# Autodesk Inventor assembly: kls15-225-m12
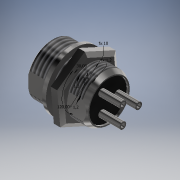
[picture p0: Inventor's stored thumbnail of the model, 180x180]
Saved by Autodesk Inventor 2019 (Build 230136000, 136)
## iProperties
Created: 2019-07-16
Part Number: kls15-225-m12
Material: Типовые
Document SubType Name: Assembly
Designer: Boss
Mass: 8.12231 g
Surface Area: 21.6045 cm^2
Volume: 1.41247 cm^3
Density: 5.75041 g/cm^3
Author: Boss
## Documents named in this file (5)
- C:\Users\Surflay\Desktop\Университет\ПД\Модели\3-pin\3-pin.iam
- C:\Users\Surflay\Desktop\Университет\ПД\Модели\3-pin\корпус разъема.ipt
- C:\Users\Surflay\Desktop\Университет\ПД\Модели\3-pin\каркас.ipt
- C:\Users\Surflay\Desktop\Университет\ПД\Модели\3-pin\kls_pin.ipt
- C:\Users\Surflay\Desktop\Университет\ПД\Модели\3-pin\гайка.ipt
## Components (6 placed, 4 different names)
1. корпус разъема:1 — Совмещение:1, Совмещение:2, Угол:1, Вставка:1, Угол:2, Вставка:4
2. каркас:1 — Вставка:1, Угол:2, Вставка:7, Вставка:8, Вставка:9
3. kls_pin:1 — Вставка:8
4. kls_pin:2 — Вставка:7
5. гайка:1 — Вставка:4
6. kls_pin:3 — Вставка:9
## Relationships (9: Insert 5, Mate 2, Angle 2)
- Совмещение:1 [Mate]: корпус разъема:1
- Совмещение:2 [Mate]: корпус разъема:1
- Угол:1 [Angle] (0 deg): корпус разъема:1
- Вставка:1 [Insert]: корпус разъема:1 ↔ каркас:1
- Угол:2 [Angle] (90 deg): корпус разъема:1 ↔ каркас:1
- Вставка:4 [Insert] (1 mm): корпус разъема:1 ↔ гайка:1
- Вставка:7 [Insert]: каркас:1 ↔ kls_pin:2
- Вставка:8 [Insert]: каркас:1 ↔ kls_pin:1
- Вставка:9 [Insert]: каркас:1 ↔ kls_pin:3
